# Autodesk Inventor assembly: end section
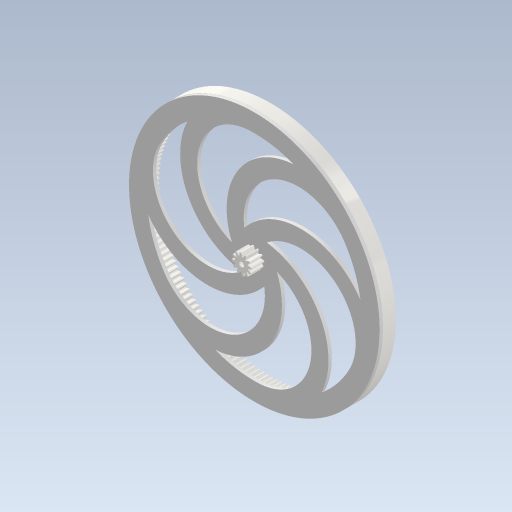
[picture p0: Inventor's stored thumbnail of the model, 512x512]
Saved by Autodesk Inventor 2023 (Build 270158000, 158)
## iProperties
Created: 2023-03-30
Part Number: end section
Document SubType Name: Assembly
Designer: dverd
Author: dverd
## Documents named in this file (4)
- C:\Users\dverd\OneDrive\Documents\ME\ME 354\turbine lab 2.0\CAD\end section.iam
- C:\Users\dverd\OneDrive\Documents\ME\ME 354\turbine lab 2.0\CAD\internal gear.ipt
- C:\Users\dverd\OneDrive\Documents\ME\ME 354\turbine lab 2.0\CAD\gear backing end.ipt
- C:\Users\dverd\OneDrive\Documents\ME\ME 354\turbine lab 2.0\CAD\small gear.ipt
## Components (3 placed, 3 different names)
1. Spur Gear2:1 — Mate:2, Mate:3
2. gear backing end:1 — Mate:2, Mate:3, Mate:4, Mate:5
3. Spur Gear1:1 — Mate:4, Mate:5
## Relationships (4: Mate 4)
- Mate:2: Spur Gear2:1 ↔ gear backing end:1
- Mate:3: Spur Gear2:1 ↔ gear backing end:1
- Mate:4: gear backing end:1 ↔ Spur Gear1:1
- Mate:5: gear backing end:1 ↔ Spur Gear1:1
